# Autodesk Inventor assembly: Ensamblaje_AntiguoFuncional
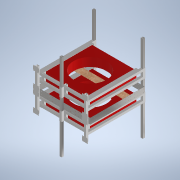
[picture p0: Inventor's stored thumbnail of the model, 180x180]
Saved by Autodesk Inventor 2020 (Build 240168000, 168)
## iProperties
Created: 2022-03-23
Part Number: Ensamblaje_AntiguoFuncional
Document SubType Name: Assembly
Designer: aarco
Author: aarco
## Documents named in this file (6)
- C:\Users\aarco\Desktop\IDOM\Ensamblaje_AntiguoFuncional.iam
- C:\Users\aarco\Desktop\IDOM\Latch.ipt
- C:\Users\aarco\Desktop\IDOM\SoporteBobina.ipt
- C:\Users\aarco\Desktop\IDOM\Madera.ipt
- C:\Users\aarco\Desktop\IDOM\Bobina.ipt
- C:\Users\aarco\Desktop\IDOM\Grid.ipt
## Components (10 placed, 5 different names)
1. Latch:1 — Rígido:1
2. SoporteBobina:1 — Coincidencia:1, Coincidencia:3, Coincidencia:4, Nivelación:1, Coincidencia:5, Coincidencia:7, Nivelación:6, Nivelación:7, Coincidencia:18, Coincidencia:19
3. Madera:1 — Rígido:1, Rígido:2, Coincidencia:13, Ángulo:1, Rígido:3, Rígido:4, Coincidencia:14, Coincidencia:15, Nivelación:8
4. Latch:2 — Rígido:2
5. Bobina:1 — Coincidencia:1, Coincidencia:3, Coincidencia:4
6. Grid:1 — Coincidencia:11, Coincidencia:14, Coincidencia:15, Nivelación:8, Coincidencia:17, Coincidencia:18
7. SoporteBobina:2 — Nivelación:6, Nivelación:7, Coincidencia:11, Coincidencia:19
8. Bobina:2
9. Latch:3 — Rígido:3
10. Latch:4 — Rígido:4
## Relationships (24: Mate 15, WeldJoint 4, Flush 4, Angle 1)
- Rígido:1 [WeldJoint]: Latch:1 ↔ Madera:1
- Rígido:2 [WeldJoint]: Madera:1 ↔ Latch:2
- Coincidencia:1 [Mate]: SoporteBobina:1 ↔ Bobina:1
- Coincidencia:3 [Mate]: SoporteBobina:1 ↔ Bobina:1
- Coincidencia:4 [Mate]: SoporteBobina:1 ↔ Bobina:1
- Nivelación:1 [Flush] (500 mm): SoporteBobina:1
- Coincidencia:5 [Mate]: SoporteBobina:1
- Coincidencia:7 [Mate]: SoporteBobina:1
- [Mate]: SoporteBobina:2 ↔ Bobina:2
- [Mate]: SoporteBobina:2 ↔ Bobina:2
- [Mate]: SoporteBobina:2 ↔ Bobina:2
- Nivelación:6 [Flush]: SoporteBobina:1 ↔ SoporteBobina:2
- Nivelación:7 [Flush]: SoporteBobina:1 ↔ SoporteBobina:2
- Coincidencia:11 [Mate]: Grid:1 ↔ SoporteBobina:2
- Coincidencia:13 [Mate]: Madera:1
- Ángulo:1 [Angle] (0 deg): Madera:1
- Rígido:3 [WeldJoint]: Madera:1 ↔ Latch:3
- Rígido:4 [WeldJoint]: Madera:1 ↔ Latch:4
- Coincidencia:14 [Mate]: Madera:1 ↔ Grid:1
- Coincidencia:15 [Mate] (400 mm): Madera:1 ↔ Grid:1
- Nivelación:8 [Flush]: Madera:1 ↔ Grid:1
- Coincidencia:17 [Mate]: Grid:1
- Coincidencia:18 [Mate] (800 mm): SoporteBobina:1 ↔ Grid:1
- Coincidencia:19 [Mate]: SoporteBobina:1 ↔ SoporteBobina:2
## Named parameters: d28_d9 = 0 mm, d29_d11 = 0 mm, d30_d15 = 0 mm, d31_d16 = 1000 mm, d32_d17 = 0 mm
